# Autodesk Inventor assembly: Link_3
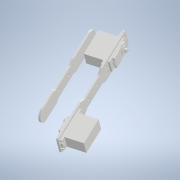
[picture p0: Inventor's stored thumbnail of the model, 180x180]
Saved by Autodesk Inventor 2022 (Build 260153000, 153)
## iProperties
Created: 2021-09-23
Part Number: Link_3
Document SubType Name: Assembly
Designer: Administrador
Author: Administrador
## Documents named in this file (4)
- C:\Users\Administrador\Desktop\Octavo Semestre\Robótica Industrial\Robot\Links\Link_3.iam
- C:\Users\Administrador\Desktop\Octavo Semestre\Robótica Industrial\Robot\Cuerpo\PartesCuerpo\Brazo2Izquierda.ipt
- C:\Users\Administrador\Desktop\Octavo Semestre\Robótica Industrial\Robot\Cuerpo\PartesCuerpo\Brazo2Derecha.ipt
- C:\Users\Administrador\Desktop\Octavo Semestre\Robótica Industrial\Robot\Cuerpo\PartesCuerpo\Motor Mg995.ipt
## Components (4 placed, 3 different names)
1. Brazo2Izquierda:1
2. Brazo2Derecha:1
3. Motor Mg995:1
4. Motor Mg995:2
## Relationships (7: Mate 7)
- [Mate]: Brazo2Derecha:1 ↔ Motor Mg995:1
- [Mate]: Brazo2Derecha:1 ↔ Motor Mg995:1
- [Mate]: Brazo2Derecha:1 ↔ Motor Mg995:1
- [Mate]: Brazo2Izquierda:1 ↔ Brazo2Derecha:1
- [Mate]: Brazo2Derecha:1 ↔ Motor Mg995:2
- [Mate]: Brazo2Derecha:1 ↔ Motor Mg995:2
- [Mate]: Brazo2Derecha:1 ↔ Motor Mg995:2
